# Autodesk Inventor assembly: PCB Component
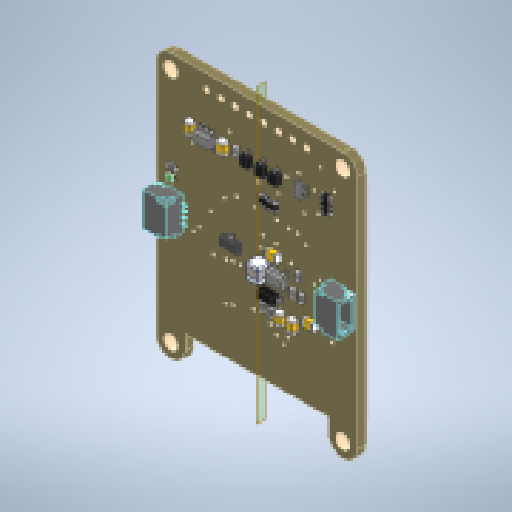
[picture p0: Inventor's stored thumbnail of the model, 512x512]
Saved by Autodesk Inventor 2023 (Build 270158000, 158)
## iProperties
Created: 2023-06-03
Part Number: PCB Component
Document SubType Name: Assembly
Designer: jeffb
Author: jeffb
## Documents named in this file (15)
- F:\OneDrive\Documents\Inventor\ELS\1.5 inch oled\PCB Component.iam
- F:\OneDrive\Documents\Inventor\ELS\1.5 inch oled\Board.ipt
- F:\OneDrive\Documents\Inventor\ELS\1.5 inch oled\0805-NO.ipt
- F:\OneDrive\Documents\Inventor\ELS\1.5 inch oled\SOT23-5.ipt
- F:\OneDrive\Documents\Inventor\ELS\1.5 inch oled\0603-NO.ipt
- F:\OneDrive\Documents\Inventor\ELS\1.5 inch oled\RESPACK_4X0603.ipt
- F:\OneDrive\Documents\Inventor\ELS\1.5 inch oled\SOT363.ipt
- F:\OneDrive\Documents\Inventor\ELS\1.5 inch oled\JST_SH4.ipt
- F:\OneDrive\Documents\Inventor\ELS\1.5 inch oled\CHIPLED_0603_NOOUTLINE.ipt
- F:\OneDrive\Documents\Inventor\ELS\1.5 inch oled\SOT23.ipt
- F:\OneDrive\Documents\Inventor\ELS\1.5 inch oled\SOD-323.ipt
- F:\OneDrive\Documents\Inventor\ELS\1.5 inch oled\OLED_1.5IN_128X128MONO.ipt
- F:\OneDrive\Documents\Inventor\ELS\1.5 inch oled\SOT23-5@1.ipt
- F:\OneDrive\Documents\Inventor\ELS\1.5 inch oled\INDUCTOR_1007.ipt
- F:\OneDrive\Documents\Inventor\ELS\1.5 inch oled\SOD-123.ipt
## Components (29 placed, 29 different names)
1. Board:1 — Flush:1
2. 0805-NO:C2
3. 0805-NO:C3
4. 0805-NO:C14
5. 0805-NO:C15
6. 0805-NO:C16
7. 0805-NO:C7
8. SOT23-5:U2
9. 0603-NO:C1
10. 0603-NO:R1
11. 0603-NO:R9
12. 0603-NO:C17
13. 0603-NO:R6
14. 0603-NO:R7
15. 0603-NO:C8
16. RESPACK_4X0603:R3
17. RESPACK_4X0603:R2
18. SOT363:Q2
19. JST_SH4:CONN4
20. JST_SH4:CONN1
21. CHIPLED_0603_NOOUTLINE:D1
22. SOT23:IC5
23. SOD-323:D3
24. SOD-323:D4
25. SOD-323:D5
26. OLED_1.5IN_128X128MONO:X1
27. SOT23-5@1:U3
28. INDUCTOR_1007:L1
29. SOD-123:D2
## Relationships (1: Flush 1)
- Flush:1 (-17.78 mm): Board:1
